# Autodesk Inventor assembly: Ensamblaje3
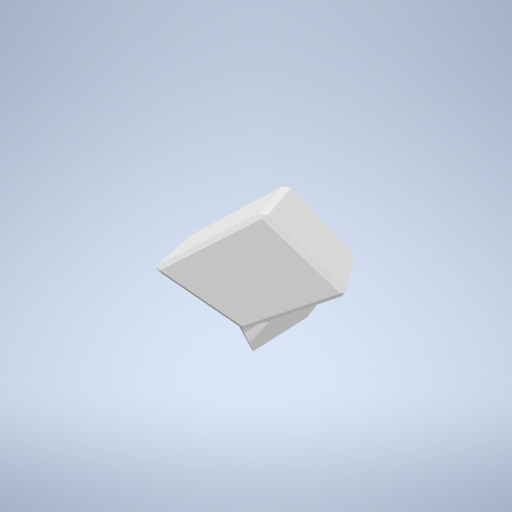
[picture p0: Inventor's stored thumbnail of the model, 512x512]
Saved by Autodesk Inventor 2024 (Build 280153000, 153)
## iProperties
Created: 2024-04-21
Part Number: Ensamblaje3
Document SubType Name: Assembly
Designer: sergi
Author: sergi
## Documents named in this file (3)
- C:\Users\sergi\OneDrive\Escritorio\proyectos\Piso\Dodecaedro\Ensamblaje3.iam
- C:\Users\sergi\OneDrive\Escritorio\proyectos\Piso\Dodecaedro\Aux2.ipt
- C:\Users\sergi\OneDrive\Escritorio\proyectos\Piso\Dodecaedro\Union.ipt
## Components (2 placed, 2 different names)
1. Aux2:1 — Coincidencia:1
2. Union:1 — Coincidencia:1
## Relationships (1: Mate 1)
- Coincidencia:1 [Mate]: Aux2:1 ↔ Union:1
